# Autodesk Inventor assembly: s-assy-shooter_frame
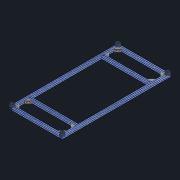
[picture p0: Inventor's stored thumbnail of the model, 180x180]
Saved by Autodesk Inventor 2022 (Build 260153000, 153)
## iProperties
Created: 2021-09-11
Part Number: s-assy-shooter_frame
Document SubType Name: Assembly
Designer: yuto6
Mass: 1668.34 g
Surface Area: 5580.12 cm^2
Volume: 592.585 cm^3
Density: 2.81536 g/cm^3
Author: yuto6
## Documents named in this file (8)
- C:\Users\yuta0\Desktop\catchrobo_shooter\s-assy-shooter_frame.iam
- C:\Users\yuta0\Desktop\catchrobo_shooter\s-assy-blacket.iam
- C:\Users\yuta0\Desktop\catchrobo_shooter\HNTC5-5.iam
- C:\Users\yuta0\Desktop\catchrobo_shooter\NFS5-2020-351.ipt
- C:\Users\yuta0\Desktop\catchrobo_shooter\NFS5-2020-805.ipt
- C:\Users\yuta0\Desktop\catchrobo_shooter\K-34.ipt
- C:\Users\yuta0\Desktop\catchrobo_shooter\HNTT5-5.ipt
- C:\Users\yuta0\Desktop\catchrobo_shooter\CB5-12.ipt
## Components (42 placed, 7 different names)
1. NFS5-2020-805:1 — メイト:1, メイト:2, フラッシュ:1, フラッシュ:2, メイト:3, フラッシュ:3, フラッシュ:4, フラッシュ:7, メイト:5, フラッシュ:8, メイト:8, メイト:15, メイト:16, メイト:17, メイト:18
2. NFS5-2020-805:2 — メイト:4, フラッシュ:5, フラッシュ:6, フラッシュ:9, メイト:9, メイト:12, フラッシュ:10, メイト:25, メイト:26, メイト:27, メイト:29, メイト:30
3. NFS5-2020-351:2 — メイト:3, フラッシュ:3, フラッシュ:4, メイト:7, メイト:10
4. s-assy-blacket:4 [sub-assembly] — フラッシュ:9, メイト:9, メイト:10
5. s-assy-blacket:2 [sub-assembly] — フラッシュ:8, メイト:7, メイト:8
6. NFS5-2020-351:3
7. s-assy-blacket:6 [sub-assembly]
8. s-assy-blacket:7 [sub-assembly]
9. NFS5-2020-351:1 — メイト:1, メイト:2, フラッシュ:1, フラッシュ:2, メイト:4, フラッシュ:5, フラッシュ:6, メイト:6, メイト:11, メイト:13, メイト:14, メイト:19, メイト:20, メイト:21, メイト:22
10. s-assy-blacket:1 [sub-assembly] — フラッシュ:7, メイト:5, メイト:6
11. s-assy-blacket:5 [sub-assembly] — メイト:11, メイト:12, フラッシュ:10
12. NFS5-2020-351:4
13. s-assy-blacket:8 [sub-assembly]
14. s-assy-blacket:9 [sub-assembly]
15. K-34:1 — メイト:25, メイト:28, メイト:29, メイト:31, メイト:32
16. HNTT5-5:1 — メイト:26, メイト:27, メイト:28, メイト:30
17. CB5-12:1 — メイト:31, メイト:32
18. K-34:2
19. HNTT5-5:2
20. CB5-12:2
21. K-34:3
22. HNTT5-5:3
23. CB5-12:3
24. K-34:4
25. HNTT5-5:4
26. CB5-12:4
27. HNTC5-5:4 [sub-assembly] — メイト:19, メイト:20, メイト:23
28. HNTC5-5:3 [sub-assembly] — メイト:21, メイト:22, メイト:24
29. HNTC5-5:1 [sub-assembly] — メイト:13, メイト:14, メイト:15, メイト:24
30. HNTC5-5:2 [sub-assembly] — メイト:16, メイト:17, メイト:18, メイト:23
31. HNTC5-5:5 [sub-assembly]
32. HNTC5-5:6 [sub-assembly]
33. HNTC5-5:7 [sub-assembly]
34. HNTC5-5:8 [sub-assembly]
35. HNTC5-5:9 [sub-assembly]
36. HNTC5-5:10 [sub-assembly]
37. HNTC5-5:11 [sub-assembly]
38. HNTC5-5:12 [sub-assembly]
39. HNTC5-5:13 [sub-assembly]
40. HNTC5-5:14 [sub-assembly]
41. HNTC5-5:15 [sub-assembly]
42. HNTC5-5:16 [sub-assembly]
## Component patterns: (2 elements, first: NFS5-2020-351:2 + s-assy-blacket:4 + s-assy-blacket:2), (2 elements, first: NFS5-2020-351:1 + s-assy-blacket:1 + s-assy-blacket:5), (4 elements, first: K-34:1 + HNTT5-5:1 + CB5-12:1), (2 elements, first: HNTC5-5:4 + HNTC5-5:3 + HNTC5-5:1 + HNTC5-5:2), (2 elements, first: HNTC5-5:9 + HNTC5-5:10 + HNTC5-5:11 + HNTC5-5:12)
## Relationships (42: Mate 32, Flush 10)
- メイト:1 [Mate]: NFS5-2020-805:1 ↔ NFS5-2020-351:1
- メイト:2 [Mate]: NFS5-2020-805:1 ↔ NFS5-2020-351:1
- フラッシュ:1 [Flush]: NFS5-2020-805:1 ↔ NFS5-2020-351:1
- フラッシュ:2 [Flush]: NFS5-2020-805:1 ↔ NFS5-2020-351:1
- メイト:3 [Mate]: NFS5-2020-805:1 ↔ NFS5-2020-351:2
- フラッシュ:3 [Flush]: NFS5-2020-805:1 ↔ NFS5-2020-351:2
- フラッシュ:4 [Flush]: NFS5-2020-805:1 ↔ NFS5-2020-351:2
- メイト:4 [Mate]: NFS5-2020-805:2 ↔ NFS5-2020-351:1
- フラッシュ:5 [Flush]: NFS5-2020-805:2 ↔ NFS5-2020-351:1
- フラッシュ:6 [Flush]: NFS5-2020-805:2 ↔ NFS5-2020-351:1
- フラッシュ:7 [Flush]: NFS5-2020-805:1 ↔ s-assy-blacket:1
- メイト:5 [Mate]: NFS5-2020-805:1 ↔ s-assy-blacket:1
- メイト:6 [Mate]: NFS5-2020-351:1 ↔ s-assy-blacket:1
- フラッシュ:8 [Flush]: NFS5-2020-805:1 ↔ s-assy-blacket:2
- メイト:7 [Mate]: NFS5-2020-351:2 ↔ s-assy-blacket:2
- メイト:8 [Mate]: NFS5-2020-805:1 ↔ s-assy-blacket:2
- フラッシュ:9 [Flush]: NFS5-2020-805:2 ↔ s-assy-blacket:4
- メイト:9 [Mate]: NFS5-2020-805:2 ↔ s-assy-blacket:4
- メイト:10 [Mate]: NFS5-2020-351:2 ↔ s-assy-blacket:4
- メイト:11 [Mate]: NFS5-2020-351:1 ↔ s-assy-blacket:5
- メイト:12 [Mate]: NFS5-2020-805:2 ↔ s-assy-blacket:5
- フラッシュ:10 [Flush]: NFS5-2020-805:2 ↔ s-assy-blacket:5
- メイト:13 [Mate]: NFS5-2020-351:1 ↔ HNTC5-5:1
- メイト:14 [Mate] (0.1 mm): NFS5-2020-351:1 ↔ HNTC5-5:1
- メイト:15 [Mate] (5 mm): NFS5-2020-805:1 ↔ HNTC5-5:1
- メイト:16 [Mate]: NFS5-2020-805:1 ↔ HNTC5-5:2
- メイト:17 [Mate] (0.1 mm): NFS5-2020-805:1 ↔ HNTC5-5:2
- メイト:18 [Mate] (-10 mm): NFS5-2020-805:1 ↔ HNTC5-5:2
- メイト:19 [Mate]: NFS5-2020-351:1 ↔ HNTC5-5:4
- メイト:20 [Mate] (0.1 mm): NFS5-2020-351:1 ↔ HNTC5-5:4
- メイト:21 [Mate] (0.1 mm): NFS5-2020-351:1 ↔ HNTC5-5:3
- メイト:22 [Mate]: NFS5-2020-351:1 ↔ HNTC5-5:3
- メイト:23 [Mate] (190 mm): HNTC5-5:4 ↔ HNTC5-5:2
- メイト:24 [Mate] (160 mm): HNTC5-5:3 ↔ HNTC5-5:1
- メイト:25 [Mate]: NFS5-2020-805:2 ↔ K-34:1
- メイト:26 [Mate]: NFS5-2020-805:2 ↔ HNTT5-5:1
- メイト:27 [Mate] (0.1 mm): NFS5-2020-805:2 ↔ HNTT5-5:1
- メイト:28 [Mate]: K-34:1 ↔ HNTT5-5:1
- メイト:29 [Mate]: NFS5-2020-805:2 ↔ K-34:1
- メイト:30 [Mate] (-10 mm): NFS5-2020-805:2 ↔ HNTT5-5:1
- メイト:31 [Mate]: K-34:1 ↔ CB5-12:1
- メイト:32 [Mate]: K-34:1 ↔ CB5-12:1
